# Autodesk Inventor assembly: ForeArm
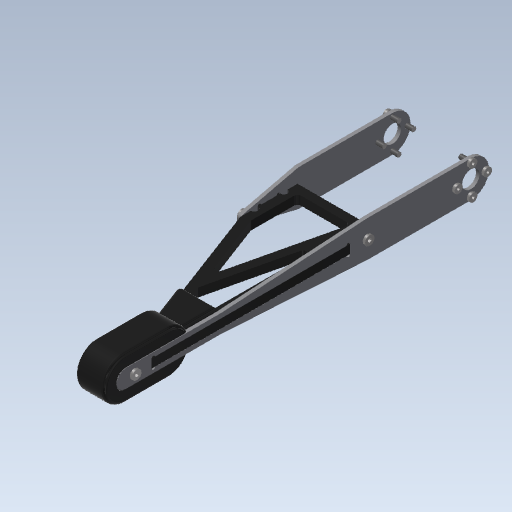
[picture p0: Inventor's stored thumbnail of the model, 512x512]
Saved by Autodesk Inventor 2020 (Build 240168000, 168)
## iProperties
Created: 2016-05-04
Part Number: ForeArm
Document SubType Name: Assembly
Designer: hiroaki
Mass: 59.7567 g
Surface Area: 275.043 cm^2
Volume: 46.6042 cm^3
Density: 1.28222 g/cm^3
Author: hiroaki
## Documents named in this file (9)
- C:\Users\Masato\Documents\Inventor\CIT Brains_Inventor\OpenPlatform_ver3_0 - Ver4_1branch\UpperBody\Arm\ForeArm.iam
- C:\Users\Masato\Documents\Inventor\CIT Brains_Inventor\OpenPlatform_ver3_0 - Ver4_1branch\UpperBody\Arm\ForeArm_outside_frame.ipt
- C:\Users\Masato\Documents\Inventor\CIT Brains_Inventor\OpenPlatform_ver3_0 - Ver4_1branch\UpperBody\Arm\ForeArm_diagonal.ipt
- C:\Users\Masato\Documents\Inventor\CIT Brains_Inventor\OpenPlatform_ver3_0 - Ver4_1branch\UpperBody\Arm\ForeArm_inside_frame.ipt
- C:\Users\Masato\Documents\Inventor\CIT Brains_Inventor\OpenPlatform_ver3_0 - Ver4_1branch\Ready_Made\Screw\M3-6.ipt
- C:\Users\Masato\Documents\Inventor\CIT Brains_Inventor\OpenPlatform_ver3_0 - Ver4_1branch\Ready_Made\Screw\M3-10.ipt
- C:\Users\Masato\Documents\Inventor\CIT Brains_Inventor\OpenPlatform_ver3_0\Ready_Made\UD-43040.ipt
- C:\Users\Masato\Documents\Inventor\CIT Brains_Inventor\OpenPlatform_ver3_0 - Ver4_1branch\UpperBody\Arm\Hand.ipt
- C:\Users\Masato\Documents\Inventor\CIT Brains_Inventor\OpenPlatform_ver3_0 - Ver4_1branch\Ready_Made\Screw\M2_6-6.ipt
## Components (17 placed, 8 different names)
1. ForeArm_diagonal:1 — メイト:1, メイト:2, フラッシュ:1, 挿入:3, 挿入:4, 挿入:5, 挿入:6, 角度:1, 挿入:12
2. ForeArm_outside_frame:1 — 挿入:3, 挿入:4, 挿入:7, 挿入:10, 挿入:13, 挿入:14, 挿入:15, 挿入:16
3. ForeArm_inside_frame:1 — 挿入:5, 挿入:6, 挿入:8, 挿入:9, 挿入:17, 挿入:18, 挿入:19, 挿入:20
4. M3-6:1 — 挿入:7
5. M3-6:2 — 挿入:8
6. M3-6:3 — 挿入:9
7. M3-10:1 — 挿入:10
8. UD-43040:1 — 挿入:11
9. Hand:1 — 角度:1, 挿入:12, 挿入:11
10. M2_6-6:1 — 挿入:16
11. M2_6-6:2 — 挿入:17
12. M2_6-6:3 — 挿入:18
13. M2_6-6:4 — 挿入:19
14. M2_6-6:5 — 挿入:20
15. M2_6-6:6 — 挿入:13
16. M2_6-6:7 — 挿入:14
17. M2_6-6:8 — 挿入:15
## Relationships (22: Insert 18, Mate 2, Flush 1, Angle 1)
- メイト:1 [Mate]: ForeArm_diagonal:1
- メイト:2 [Mate]: ForeArm_diagonal:1
- フラッシュ:1 [Flush]: ForeArm_diagonal:1
- 挿入:3 [Insert]: ForeArm_diagonal:1 ↔ ForeArm_outside_frame:1
- 挿入:4 [Insert]: ForeArm_diagonal:1 ↔ ForeArm_outside_frame:1
- 挿入:5 [Insert]: ForeArm_diagonal:1 ↔ ForeArm_inside_frame:1
- 挿入:6 [Insert]: ForeArm_diagonal:1 ↔ ForeArm_inside_frame:1
- 挿入:7 [Insert]: ForeArm_outside_frame:1 ↔ M3-6:1
- 挿入:8 [Insert]: ForeArm_inside_frame:1 ↔ M3-6:2
- 挿入:9 [Insert]: ForeArm_inside_frame:1 ↔ M3-6:3
- 挿入:10 [Insert]: ForeArm_outside_frame:1 ↔ M3-10:1
- 挿入:11 [Insert]: UD-43040:1 ↔ Hand:1
- 角度:1 [Angle] (0 deg): ForeArm_diagonal:1 ↔ Hand:1
- 挿入:12 [Insert] (0.25 mm): ForeArm_diagonal:1 ↔ Hand:1
- 挿入:13 [Insert]: ForeArm_outside_frame:1 ↔ M2_6-6:6
- 挿入:14 [Insert]: ForeArm_outside_frame:1 ↔ M2_6-6:7
- 挿入:15 [Insert]: ForeArm_outside_frame:1 ↔ M2_6-6:8
- 挿入:16 [Insert]: ForeArm_outside_frame:1 ↔ M2_6-6:1
- 挿入:17 [Insert]: ForeArm_inside_frame:1 ↔ M2_6-6:2
- 挿入:18 [Insert]: ForeArm_inside_frame:1 ↔ M2_6-6:3
- 挿入:19 [Insert]: ForeArm_inside_frame:1 ↔ M2_6-6:4
- 挿入:20 [Insert]: ForeArm_inside_frame:1 ↔ M2_6-6:5
